# Autodesk Inventor assembly: One_finger_assembly
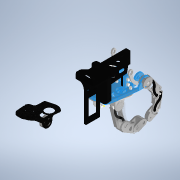
[picture p0: Inventor's stored thumbnail of the model, 180x180]
Saved by Autodesk Inventor 2020.3 (Build 243373000, 373)
## iProperties
Created: 2021-03-23
Part Number: One_finger_assembly
Document SubType Name: Assembly
Designer: sanyi
Author: sanyi
## Documents named in this file (20)
- E:\Dokumentumok\Simonyi\INDACT\Robotarm - kézfej fileok\One_finger_assembly.iam
- E:\Dokumentumok\Simonyi\INDACT\Robotarm - kézfej fileok\kéz12.0\Solid1_1.ipt
- E:\Dokumentumok\Simonyi\INDACT\Robotarm - kézfej fileok\kéz12.0\Solid4_11.ipt
- E:\Dokumentumok\Simonyi\INDACT\Robotarm - kézfej fileok\kéz12.0\Solid1.ipt
- E:\Dokumentumok\Simonyi\INDACT\Robotarm - kézfej fileok\kéz12.0\Solid1_MIR1.ipt
- E:\Dokumentumok\Simonyi\INDACT\Robotarm - kézfej fileok\kéz12.0\Solid2.ipt
- E:\Dokumentumok\Simonyi\INDACT\Robotarm - kézfej fileok\kéz12.0\Solid2_MIR2.ipt
- E:\Dokumentumok\Simonyi\INDACT\Robotarm - kézfej fileok\kéz12.0\Solid3.ipt
- E:\Dokumentumok\Simonyi\INDACT\Robotarm - kézfej fileok\kéz12.0\Solid3_MIR2.ipt
- E:\Dokumentumok\Simonyi\INDACT\Robotarm - kézfej fileok\kéz12.0\Solid5.ipt
- E:\Dokumentumok\Simonyi\INDACT\Robotarm - kézfej fileok\kéz12.0\Solid6.ipt
- E:\Dokumentumok\Simonyi\INDACT\Robotarm - kézfej fileok\kéz12.0\Solid3_1.ipt
- E:\Dokumentumok\Simonyi\INDACT\Robotarm - kézfej fileok\kéz12.0\Solid4_1.ipt
- E:\Dokumentumok\Simonyi\INDACT\Robotarm - kézfej fileok\kéz12.0\Solid12.ipt
- E:\Dokumentumok\Simonyi\INDACT\Robotarm - kézfej fileok\kéz12.0\Solid1_11.ipt
- E:\Dokumentumok\Simonyi\INDACT\Robotarm - kézfej fileok\kéz12.0\Solid2_1.ipt
- E:\Dokumentumok\Simonyi\INDACT\Robotarm - kézfej fileok\kéz12.0\Solid13_mother_m2_5.ipt
- E:\Dokumentumok\Simonyi\INDACT\Robotarm - kézfej fileok\kéz12.0\Part2.ipt
- E:\Dokumentumok\Simonyi\INDACT\Robotarm - kézfej fileok\kéz12.0\Part6.ipt
- E:\Dokumentumok\Simonyi\INDACT\Robotarm - kézfej fileok\kéz12.0\Solid3_1v2.ipt
## Components (46 placed, 19 different names)
1. Solid1_1:1 — Mate:1, Mate:2, Mate:3, Mate:4, Mate:5, Mate:6, Insert:7, Insert:11, Insert:39, Insert:42, Insert:43, Mate:16, Insert:44, Insert:46, Insert:62, Insert:63, Insert:67, Insert:68, Insert:69, Insert:72
2. Solid4_11:1 — Mate:4, Mate:5, Mate:6, Insert:15
3. Solid1:1 — Mate:7, Insert:11, Insert:12, Insert:13, Angle:1, Insert:33, Insert:47, Insert:48
4. Solid1_MIR1:1 — Mate:7, Angle:1, Insert:15, Insert:16
5. Solid2:1 — Insert:6, Mate:8, Insert:12, Insert:14, Angle:2, Insert:32
6. Solid2_MIR2:1 — Mate:8, Angle:2, Insert:16, Insert:17
7. Solid3:1 — Insert:4, Mate:9, Insert:14, Angle:3, Insert:31
8. Solid3_MIR2:1 — Mate:9, Angle:3, Insert:17
9. Solid5:1 — Insert:6, Insert:7
10. Solid6:1 — Insert:4, Insert:13
11. Solid3_1:1 — Mate:10, Mate:11, Mate:12
12. Solid4_1:1 — Mate:10, Mate:11, Mate:12
13. Solid1:2 — Mate:13, Angle:4, Insert:29, Insert:66
14. Solid1_MIR1:2 — Insert:22, Insert:26, Mate:13, Angle:4, Insert:36, Insert:70
15. Solid2:2 — Mate:14, Angle:5, Insert:29, Insert:30
16. Solid2_MIR2:2 — Insert:22, Insert:23, Insert:25, Mate:14, Angle:5, Insert:35
17. Solid3:2 — Mate:15, Angle:6, Insert:30
18. Solid3_MIR2:2 — Insert:25, Insert:27, Mate:15, Angle:6, Insert:34
19. Solid5:2 — Insert:23, Insert:71
20. Solid6:2 — Insert:26, Insert:27
21. Solid12:1 — Insert:31
22. Solid12:2 — Insert:32
23. Solid12:3 — Insert:33
24. Solid12:4 — Insert:34
25. Solid12:5 — Insert:35
26. Solid12:6 — Insert:36, Insert:66
27. Solid1_11:1 — Insert:45, Insert:46
28. Solid2_1:1 — Insert:39, Insert:44, Insert:45
29. Solid13_mother_m2_5:1 — Insert:43
30. Solid13_mother_m2_5:2 — Insert:42
31. Solid13_mother_m2_5:3 — Mate:16
32. Solid13_mother_m2_5:4 — Insert:47
33. Part2:1 — Insert:64
34. Part6:1 — Insert:48
35. Solid1:3 — Mate:17, Flush:1
36. Solid2:3
37. Solid3:3
38. Solid5:3 — Insert:63
39. Solid6:3
40. Solid12:7
41. Solid12:8
42. Solid12:9 — Insert:61
43. Solid1_MIR1:3 — Mate:17, Flush:1, Insert:61, Insert:62, Insert:64, Insert:65
44. Solid13_mother_m2_5:6 — Insert:65
45. Solid3_1v2:1 — Insert:67, Insert:68, Insert:69, Insert:70, Insert:71
46. Solid13_mother_m2_5:7 — Insert:72
## Relationships (75: Insert 51, Mate 17, Angle 6, Flush 1)
- Mate:1: Solid1_1:1
- Mate:2: Solid1_1:1
- Mate:3: Solid1_1:1
- Mate:4: Solid1_1:1 ↔ Solid4_11:1
- Mate:5 (0.25 mm): Solid1_1:1 ↔ Solid4_11:1
- Mate:6 (0.25 mm): Solid1_1:1 ↔ Solid4_11:1
- Insert:4 (3.5 mm): Solid3:1 ↔ Solid6:1
- Insert:6 (3.5 mm): Solid2:1 ↔ Solid5:1
- Insert:7 (0.5 mm): Solid1_1:1 ↔ Solid5:1
- Mate:7: Solid1:1 ↔ Solid1_MIR1:1
- Mate:8: Solid2:1 ↔ Solid2_MIR2:1
- Mate:9: Solid3:1 ↔ Solid3_MIR2:1
- Insert:11 (0.2 mm): Solid1_1:1 ↔ Solid1:1
- Insert:12 (0.2 mm): Solid1:1 ↔ Solid2:1
- Insert:13 (0.5 mm): Solid1:1 ↔ Solid6:1
- Insert:14 (0.2 mm): Solid2:1 ↔ Solid3:1
- Angle:1 (0 deg): Solid1:1 ↔ Solid1_MIR1:1
- Insert:15 (0.2 mm): Solid4_11:1 ↔ Solid1_MIR1:1
- Angle:2 (0 deg): Solid2:1 ↔ Solid2_MIR2:1
- Angle:3 (0 deg): Solid3:1 ↔ Solid3_MIR2:1
- Insert:16 (0.2 mm): Solid1_MIR1:1 ↔ Solid2_MIR2:1
- Insert:17 (0.2 mm): Solid2_MIR2:1 ↔ Solid3_MIR2:1
- Mate:10: Solid3_1:1 ↔ Solid4_1:1
- Mate:11 (0.25 mm): Solid3_1:1 ↔ Solid4_1:1
- Mate:12 (0.25 mm): Solid3_1:1 ↔ Solid4_1:1
- Insert:22 (0.2 mm): Solid1_MIR1:2 ↔ Solid2_MIR2:2
- Insert:23 (3.5 mm): Solid2_MIR2:2 ↔ Solid5:2
- Insert:25 (0.2 mm): Solid2_MIR2:2 ↔ Solid3_MIR2:2
- Insert:26 (0.5 mm): Solid1_MIR1:2 ↔ Solid6:2
- Insert:27 (3.5 mm): Solid3_MIR2:2 ↔ Solid6:2
- Mate:13: Solid1:2 ↔ Solid1_MIR1:2
- Mate:14: Solid2:2 ↔ Solid2_MIR2:2
- Mate:15: Solid3:2 ↔ Solid3_MIR2:2
- Angle:4 (0 deg): Solid1:2 ↔ Solid1_MIR1:2
- Angle:5 (0 deg): Solid2:2 ↔ Solid2_MIR2:2
- Angle:6 (0 deg): Solid3:2 ↔ Solid3_MIR2:2
- Insert:29 (0.2 mm): Solid1:2 ↔ Solid2:2
- Insert:30 (0.2 mm): Solid2:2 ↔ Solid3:2
- Insert:31 (0.1 mm): Solid3:1 ↔ Solid12:1
- Insert:32 (0.1 mm): Solid2:1 ↔ Solid12:2
- Insert:33 (0.1 mm): Solid1:1 ↔ Solid12:3
- Insert:34 (0.1 mm): Solid3_MIR2:2 ↔ Solid12:4
- Insert:35 (0.1 mm): Solid2_MIR2:2 ↔ Solid12:5
- Insert:36 (0.1 mm): Solid1_MIR1:2 ↔ Solid12:6
- Insert:39: Solid1_1:1 ↔ Solid2_1:1
- Insert:42: Solid1_1:1 ↔ Solid13_mother_m2_5:2
- Insert:43: Solid1_1:1 ↔ Solid13_mother_m2_5:1
- Mate:16: Solid1_1:1 ↔ Solid13_mother_m2_5:3
- Insert:44: Solid1_1:1 ↔ Solid2_1:1
- Insert:45: Solid1_11:1 ↔ Solid2_1:1
- Insert:46: Solid1_1:1 ↔ Solid1_11:1
- Insert:47: Solid1:1 ↔ Solid13_mother_m2_5:4
- Insert:48 (0.2 mm): Solid1:1 ↔ Part6:1
- [Insert] (3.5 mm): Solid3:3 ↔ Solid6:3
- [Insert] (3.5 mm): Solid2:3 ↔ Solid5:3
- [Insert] (0.2 mm): Solid1:3 ↔ Solid2:3
- [Insert] (0.5 mm): Solid1:3 ↔ Solid6:3
- [Insert] (0.2 mm): Solid2:3 ↔ Solid3:3
- [Insert] (0.1 mm): Solid3:3 ↔ Solid12:7
- [Insert] (0.1 mm): Solid2:3 ↔ Solid12:8
- [Insert] (0.1 mm): Solid1:3 ↔ Solid12:9
- Mate:17: Solid1:3 ↔ Solid1_MIR1:3
- Flush:1: Solid1:3 ↔ Solid1_MIR1:3
- Insert:61 (0.1 mm): Solid12:9 ↔ Solid1_MIR1:3
- Insert:62 (0.2 mm): Solid1_1:1 ↔ Solid1_MIR1:3
- Insert:63 (0.5 mm): Solid1_1:1 ↔ Solid5:3
- Insert:64 (0.2 mm): Part2:1 ↔ Solid1_MIR1:3
- Insert:65: Solid1_MIR1:3 ↔ Solid13_mother_m2_5:6
- Insert:66 (0.1 mm): Solid1:2 ↔ Solid12:6
- Insert:67: Solid1_1:1 ↔ Solid3_1v2:1
- Insert:68: Solid1_1:1 ↔ Solid3_1v2:1
- Insert:69: Solid1_1:1 ↔ Solid3_1v2:1
- Insert:70 (0.2 mm): Solid1_MIR1:2 ↔ Solid3_1v2:1
- Insert:71 (0.5 mm): Solid5:2 ↔ Solid3_1v2:1
- Insert:72: Solid1_1:1 ↔ Solid13_mother_m2_5:7
## Named parameters: d84_d59 = 0.1 mm, d85_d60 = 0.1 mm, d86_d61 = 0.1 mm, d87_d11 = 3.5 mm, d88_d14 = 3.5 mm, d89_d25 = 0.2 mm, d90_d26 = 0.5 mm, d91_d27 = 0.2 mm
